# Autodesk Inventor assembly: Wheel holder
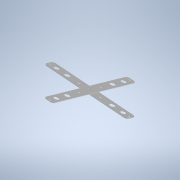
[picture p0: Inventor's stored thumbnail of the model, 180x180]
Saved by Autodesk Inventor 2020 (Build 240168000, 168)
## iProperties
Created: 2022-07-02
Part Number: Wheel holder
Document SubType Name: Assembly
Designer: karimi2
Author: karimi2
## Documents named in this file (2)
- C:\Users\karimi2\Documents\PROJECT\src\Wheel holder.iam
- C:\Users\karimi2\Documents\PROJECT\src\chassisPart1.ipt
## Components (2 placed, 1 different names)
1. chassisPart1:1 — Rigid:1
2. chassisPart1:2 — Rigid:1
## Relationships (1: WeldJoint 1)
- Rigid:1 [WeldJoint]: chassisPart1:1 ↔ chassisPart1:2
